# Autodesk Inventor assembly: CE-7.1.1
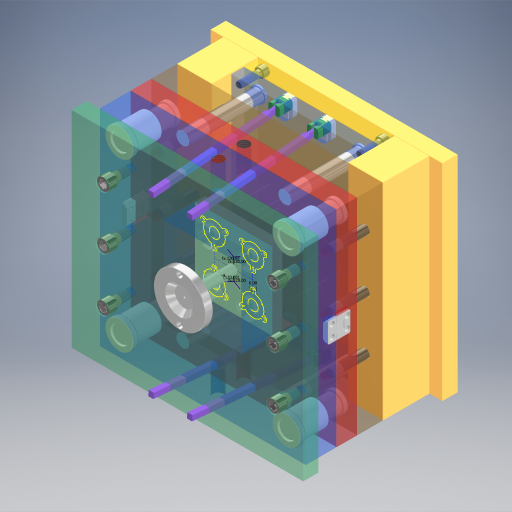
[picture p0: Inventor's stored thumbnail of the model, 512x512]
Saved by Autodesk Inventor 2024 (Build 280153000, 153)
## iProperties
Created: 2024-02-25
Part Number: CE-7.1.1
Document SubType Name: Assembly
Designer: Alex
Author: Alex
## Documents named in this file (10)
- C:\Shared\alex-bartella-schoolwork\4z03\Week 6\CE-7.1.1.iam
- C:\Shared\alex-bartella-schoolwork\4z03\Week 6\CE-7.1.1_CE-2.1.4_LY.iam
- C:\Shared\alex-bartella-schoolwork\4z03\Week 6\CE-7.1.1_Combined CV1.ipt
- C:\Shared\alex-bartella-schoolwork\4z03\Week 6\CE-7.1.1_Combined CR1.ipt
- C:\Shared\alex-bartella-schoolwork\4z03\Week 6\MB\FUTABA_SA-S 1\CE-7.1.1_MB.iam
- C:\Shared\alex-bartella-schoolwork\4z03\Week 6\CE-7.1.1_RG.ipt
- C:\Shared\alex-bartella-schoolwork\4z03\Week 6\Sprue Bushing\HASCO_Z51\CE-7.1.1_Z51-18x76-3.5.ipt
- C:\Shared\alex-bartella-schoolwork\4z03\Week 6\Locating Ring\LKM_LR\CE-7.1.1_LR-100-36.ipt
- C:\Shared\alex-bartella-schoolwork\4z03\Week 6\LS\DME_FW45 2\CE-7.1.1_LS1.iam
- C:\Shared\alex-bartella-schoolwork\4z03\Week 6\LS\DME_FW45 3\CE-7.1.1_LS2.iam
## Components (9 placed, 8 different names)
1. CE-7.1.1_CE-2.1.4_LY:1 [sub-assembly] — Flush:1, Flush:2, Flush:3, Flush:10, Flush:19, Flush:20, Flush:21, Flush:22, Flush:23, Flush:24, Mate:2, Flush:25, Flush:26, Mate:3, Flush:27, Flush:28, Mate:4, Flush:29, Flush:30, Mate:5, Flush:31, Flush:32, Flush:33, Flush:34, Flush:35, Flush:36, Flush:37, Flush:38, Flush:39, Flush:40, Flush:41, Flush:42, Flush:43, Flush:44, Flush:45, Flush:46, Flush:47, Flush:48, Flush:49, Flush:50, Flush:51, Flush:52, Flush:53, Flush:54, Flush:61, Flush:62, Flush:63, Flush:64, Flush:65, Flush:66, Flush:67, Flush:68, Flush:69, Flush:70, Flush:71, Flush:72, Flush:73, Flush:74, Flush:75, Flush:76, Flush:77, Flush:78, Flush:79, Flush:80, Flush:81, Flush:82, Flush:83, Flush:84, Flush:85, Flush:86, Flush:87, Flush:88, Flush:89, Flush:90, Flush:91, Flush:92, Flush:93, Flush:94, Flush:95, Flush:96
2. CE-7.1.1_Combined CV1:1 — Flush:4, Flush:5, Flush:6, Flush:55, Flush:56, Flush:57
3. CE-7.1.1_Combined CR1:1 — Flush:7, Flush:8, Flush:9, Flush:58, Flush:59, Flush:60, Flush:100
4. CE-7.1.1_MB:1 [sub-assembly] — Flush:10, Mate:1, Angle:1, Flush:19, Flush:20, Flush:21, Flush:22, Flush:23, Flush:24, Mate:2, Flush:25, Flush:26, Mate:3, Flush:27, Flush:28, Mate:4, Flush:29, Flush:30, Mate:5, Flush:31, Flush:32, Flush:33, Flush:34, Flush:35, Flush:36, Flush:37, Flush:38, Flush:39, Flush:40, Flush:41, Flush:42, Flush:43, Flush:44, Flush:45, Flush:46, Flush:47, Flush:48, Flush:49, Flush:50, Flush:51, Flush:52, Flush:53, Flush:54, Flush:55, Flush:56, Flush:57, Flush:58, Flush:59, Flush:60, Flush:61, Flush:62, Flush:63, Flush:64, Flush:65, Flush:66, Flush:67, Flush:68, Flush:69, Flush:70, Flush:71, Flush:72, Flush:73, Flush:74, Flush:75, Flush:76, Flush:77, Flush:78, Flush:79, Flush:80, Flush:81, Flush:82, Flush:83, Flush:84, Flush:85, Flush:86, Flush:87, Flush:88, Flush:89, Flush:90, Flush:91, Flush:92, Flush:93, Flush:94, Flush:95, Flush:96, Mate:6, Mate:8, Mate:10, Flush:102, Flush:103, Mate:12, Flush:104, Flush:105
5. CE-7.1.1_RG:1 — Flush:97, Flush:98, Flush:99, Flush:101, Mate:7
6. CE-7.1.1_Z51-18x76-3.5:1 — Mate:6, Mate:7, Mate:9
7. CE-7.1.1_LR-100-36:1 — Mate:8, Mate:9
8. CE-7.1:1 [sub-assembly] — Mate:10, Flush:102, Mate:11, Flush:103
9. CE-7.1:2 [sub-assembly] — Mate:12, Flush:104, Mate:13, Flush:105
## Relationships (111: Flush 97, Mate 13, Angle 1)
- Flush:1: CE-7.1.1_CE-2.1.4_LY:1
- Flush:2: CE-7.1.1_CE-2.1.4_LY:1
- Flush:3: CE-7.1.1_CE-2.1.4_LY:1
- Flush:4: CE-7.1.1_Combined CV1:1
- Flush:5: CE-7.1.1_Combined CV1:1
- Flush:6: CE-7.1.1_Combined CV1:1
- Flush:7: CE-7.1.1_Combined CR1:1
- Flush:8: CE-7.1.1_Combined CR1:1
- Flush:9: CE-7.1.1_Combined CR1:1
- Flush:10 (60 mm): CE-7.1.1_CE-2.1.4_LY:1 ↔ CE-7.1.1_MB:1
- Mate:1: CE-7.1.1_MB:1
- Angle:1 (0 deg): CE-7.1.1_MB:1
- Flush:19: CE-7.1.1_CE-2.1.4_LY:1 ↔ CE-7.1.1_MB:1
- Flush:20: CE-7.1.1_CE-2.1.4_LY:1 ↔ CE-7.1.1_MB:1
- Flush:21: CE-7.1.1_CE-2.1.4_LY:1 ↔ CE-7.1.1_MB:1
- Flush:22: CE-7.1.1_CE-2.1.4_LY:1 ↔ CE-7.1.1_MB:1
- Flush:23: CE-7.1.1_CE-2.1.4_LY:1 ↔ CE-7.1.1_MB:1
- Flush:24: CE-7.1.1_CE-2.1.4_LY:1 ↔ CE-7.1.1_MB:1
- Mate:2: CE-7.1.1_CE-2.1.4_LY:1 ↔ CE-7.1.1_MB:1
- Flush:25: CE-7.1.1_CE-2.1.4_LY:1 ↔ CE-7.1.1_MB:1
- Flush:26: CE-7.1.1_CE-2.1.4_LY:1 ↔ CE-7.1.1_MB:1
- Mate:3: CE-7.1.1_CE-2.1.4_LY:1 ↔ CE-7.1.1_MB:1
- Flush:27: CE-7.1.1_CE-2.1.4_LY:1 ↔ CE-7.1.1_MB:1
- Flush:28: CE-7.1.1_CE-2.1.4_LY:1 ↔ CE-7.1.1_MB:1
- Mate:4: CE-7.1.1_CE-2.1.4_LY:1 ↔ CE-7.1.1_MB:1
- Flush:29: CE-7.1.1_CE-2.1.4_LY:1 ↔ CE-7.1.1_MB:1
- Flush:30: CE-7.1.1_CE-2.1.4_LY:1 ↔ CE-7.1.1_MB:1
- Mate:5: CE-7.1.1_CE-2.1.4_LY:1 ↔ CE-7.1.1_MB:1
- Flush:31: CE-7.1.1_CE-2.1.4_LY:1 ↔ CE-7.1.1_MB:1
- Flush:32: CE-7.1.1_CE-2.1.4_LY:1 ↔ CE-7.1.1_MB:1
- Flush:33: CE-7.1.1_CE-2.1.4_LY:1 ↔ CE-7.1.1_MB:1
- Flush:34: CE-7.1.1_CE-2.1.4_LY:1 ↔ CE-7.1.1_MB:1
- Flush:35: CE-7.1.1_CE-2.1.4_LY:1 ↔ CE-7.1.1_MB:1
- Flush:36: CE-7.1.1_CE-2.1.4_LY:1 ↔ CE-7.1.1_MB:1
- Flush:37: CE-7.1.1_CE-2.1.4_LY:1 ↔ CE-7.1.1_MB:1
- Flush:38: CE-7.1.1_CE-2.1.4_LY:1 ↔ CE-7.1.1_MB:1
- Flush:39: CE-7.1.1_CE-2.1.4_LY:1 ↔ CE-7.1.1_MB:1
- Flush:40: CE-7.1.1_CE-2.1.4_LY:1 ↔ CE-7.1.1_MB:1
- Flush:41: CE-7.1.1_CE-2.1.4_LY:1 ↔ CE-7.1.1_MB:1
- Flush:42: CE-7.1.1_CE-2.1.4_LY:1 ↔ CE-7.1.1_MB:1
- Flush:43: CE-7.1.1_CE-2.1.4_LY:1 ↔ CE-7.1.1_MB:1
- Flush:44: CE-7.1.1_CE-2.1.4_LY:1 ↔ CE-7.1.1_MB:1
- Flush:45: CE-7.1.1_CE-2.1.4_LY:1 ↔ CE-7.1.1_MB:1
- Flush:46: CE-7.1.1_CE-2.1.4_LY:1 ↔ CE-7.1.1_MB:1
- Flush:47: CE-7.1.1_CE-2.1.4_LY:1 ↔ CE-7.1.1_MB:1
- Flush:48: CE-7.1.1_CE-2.1.4_LY:1 ↔ CE-7.1.1_MB:1
- Flush:49: CE-7.1.1_CE-2.1.4_LY:1 ↔ CE-7.1.1_MB:1
- Flush:50: CE-7.1.1_CE-2.1.4_LY:1 ↔ CE-7.1.1_MB:1
- Flush:51: CE-7.1.1_CE-2.1.4_LY:1 ↔ CE-7.1.1_MB:1
- Flush:52: CE-7.1.1_CE-2.1.4_LY:1 ↔ CE-7.1.1_MB:1
- Flush:53: CE-7.1.1_CE-2.1.4_LY:1 ↔ CE-7.1.1_MB:1
- Flush:54: CE-7.1.1_CE-2.1.4_LY:1 ↔ CE-7.1.1_MB:1
- Flush:55: CE-7.1.1_Combined CV1:1 ↔ CE-7.1.1_MB:1
- Flush:56: CE-7.1.1_Combined CV1:1 ↔ CE-7.1.1_MB:1
- Flush:57: CE-7.1.1_Combined CV1:1 ↔ CE-7.1.1_MB:1
- Flush:58: CE-7.1.1_Combined CR1:1 ↔ CE-7.1.1_MB:1
- Flush:59: CE-7.1.1_Combined CR1:1 ↔ CE-7.1.1_MB:1
- Flush:60: CE-7.1.1_Combined CR1:1 ↔ CE-7.1.1_MB:1
- Flush:61: CE-7.1.1_CE-2.1.4_LY:1 ↔ CE-7.1.1_MB:1
- Flush:62: CE-7.1.1_CE-2.1.4_LY:1 ↔ CE-7.1.1_MB:1
- Flush:63: CE-7.1.1_CE-2.1.4_LY:1 ↔ CE-7.1.1_MB:1
- Flush:64: CE-7.1.1_CE-2.1.4_LY:1 ↔ CE-7.1.1_MB:1
- Flush:65: CE-7.1.1_CE-2.1.4_LY:1 ↔ CE-7.1.1_MB:1
- Flush:66: CE-7.1.1_CE-2.1.4_LY:1 ↔ CE-7.1.1_MB:1
- Flush:67: CE-7.1.1_CE-2.1.4_LY:1 ↔ CE-7.1.1_MB:1
- Flush:68: CE-7.1.1_CE-2.1.4_LY:1 ↔ CE-7.1.1_MB:1
- Flush:69: CE-7.1.1_CE-2.1.4_LY:1 ↔ CE-7.1.1_MB:1
- Flush:70: CE-7.1.1_CE-2.1.4_LY:1 ↔ CE-7.1.1_MB:1
- Flush:71: CE-7.1.1_CE-2.1.4_LY:1 ↔ CE-7.1.1_MB:1
- Flush:72: CE-7.1.1_CE-2.1.4_LY:1 ↔ CE-7.1.1_MB:1
- Flush:73: CE-7.1.1_CE-2.1.4_LY:1 ↔ CE-7.1.1_MB:1
- Flush:74: CE-7.1.1_CE-2.1.4_LY:1 ↔ CE-7.1.1_MB:1
- Flush:75: CE-7.1.1_CE-2.1.4_LY:1 ↔ CE-7.1.1_MB:1
- Flush:76: CE-7.1.1_CE-2.1.4_LY:1 ↔ CE-7.1.1_MB:1
- Flush:77: CE-7.1.1_CE-2.1.4_LY:1 ↔ CE-7.1.1_MB:1
- Flush:78: CE-7.1.1_CE-2.1.4_LY:1 ↔ CE-7.1.1_MB:1
- Flush:79: CE-7.1.1_CE-2.1.4_LY:1 ↔ CE-7.1.1_MB:1
- Flush:80: CE-7.1.1_CE-2.1.4_LY:1 ↔ CE-7.1.1_MB:1
- Flush:81: CE-7.1.1_CE-2.1.4_LY:1 ↔ CE-7.1.1_MB:1
- Flush:82: CE-7.1.1_CE-2.1.4_LY:1 ↔ CE-7.1.1_MB:1
- Flush:83: CE-7.1.1_CE-2.1.4_LY:1 ↔ CE-7.1.1_MB:1
- Flush:84: CE-7.1.1_CE-2.1.4_LY:1 ↔ CE-7.1.1_MB:1
- Flush:85: CE-7.1.1_CE-2.1.4_LY:1 ↔ CE-7.1.1_MB:1
- Flush:86: CE-7.1.1_CE-2.1.4_LY:1 ↔ CE-7.1.1_MB:1
- Flush:87: CE-7.1.1_CE-2.1.4_LY:1 ↔ CE-7.1.1_MB:1
- Flush:88: CE-7.1.1_CE-2.1.4_LY:1 ↔ CE-7.1.1_MB:1
- Flush:89: CE-7.1.1_CE-2.1.4_LY:1 ↔ CE-7.1.1_MB:1
- Flush:90: CE-7.1.1_CE-2.1.4_LY:1 ↔ CE-7.1.1_MB:1
- Flush:91: CE-7.1.1_CE-2.1.4_LY:1 ↔ CE-7.1.1_MB:1
- Flush:92: CE-7.1.1_CE-2.1.4_LY:1 ↔ CE-7.1.1_MB:1
- Flush:93: CE-7.1.1_CE-2.1.4_LY:1 ↔ CE-7.1.1_MB:1
- Flush:94: CE-7.1.1_CE-2.1.4_LY:1 ↔ CE-7.1.1_MB:1
- Flush:95: CE-7.1.1_CE-2.1.4_LY:1 ↔ CE-7.1.1_MB:1
- Flush:96: CE-7.1.1_CE-2.1.4_LY:1 ↔ CE-7.1.1_MB:1
- Flush:97: CE-7.1.1_RG:1
- Flush:98: CE-7.1.1_RG:1
- Flush:99: CE-7.1.1_RG:1
- Flush:100: CE-7.1.1_Combined CR1:1
- Flush:101: CE-7.1.1_RG:1
- Mate:6 (-12.5 mm): CE-7.1.1_MB:1 ↔ CE-7.1.1_Z51-18x76-3.5:1
- Mate:7: CE-7.1.1_RG:1 ↔ CE-7.1.1_Z51-18x76-3.5:1
- Mate:8: CE-7.1.1_MB:1 ↔ CE-7.1.1_LR-100-36:1
- Mate:9: CE-7.1.1_Z51-18x76-3.5:1 ↔ CE-7.1.1_LR-100-36:1
- Mate:10: CE-7.1.1_MB:1 ↔ CE-7.1:1
- Flush:102: CE-7.1.1_MB:1 ↔ CE-7.1:1
- Mate:11: CE-7.1:1
- Flush:103: CE-7.1.1_MB:1 ↔ CE-7.1:1
- Mate:12: CE-7.1.1_MB:1 ↔ CE-7.1:2
- Flush:104: CE-7.1.1_MB:1 ↔ CE-7.1:2
- Mate:13: CE-7.1:2
- Flush:105: CE-7.1.1_MB:1 ↔ CE-7.1:2
